# Autodesk Inventor assembly: vtx antanna pre assem 1
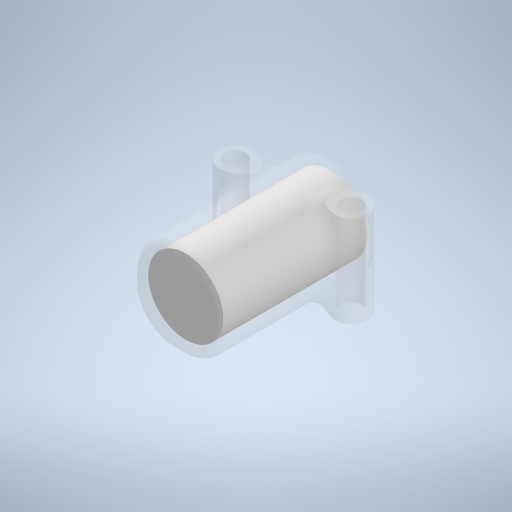
[picture p0: Inventor's stored thumbnail of the model, 512x512]
Saved by Autodesk Inventor 2023 (Build 270158000, 158)
## iProperties
Created: 2023-01-23
Part Number: vtx antanna pre assem 1
Document SubType Name: Assembly
Designer: Steven
Author: Steven
## Documents named in this file (4)
- Y:\FPV drone stuff\0 Street League\Frames\experimental-quad-frames\Nightstick MAX\3D prints\assems for derivs\vtx antanna pre assem 1.iam
- Y:\FPV drone stuff\0 Street League\Frames\experimental-quad-frames\Nightstick MAX\quad parts\SMA whip end.ipt
- Y:\FPV drone stuff\0 Street League\Frames\experimental-quad-frames\Nightstick MAX\3D prints\4700uF cap holder.ipt
- Y:\FPV drone stuff\0 Street League\Frames\experimental-quad-frames\Nightstick MAX\quad parts\4700uF cap.ipt
## Components (3 placed, 3 different names)
1. SMA whip end:1 — Mate:1, Flush:1, Flush:2, Flush:3, Angle:1
2. 4700uF cap holder:1 — Mate:1, Angle:1, Mate:2, Mate:3
3. 4700uF cap:1 — Mate:2, Mate:3
## Relationships (7: Mate 3, Flush 3, Angle 1)
- Mate:1: SMA whip end:1 ↔ 4700uF cap holder:1
- Flush:1: SMA whip end:1
- Flush:2: SMA whip end:1
- Flush:3: SMA whip end:1
- Angle:1 (0 deg): SMA whip end:1 ↔ 4700uF cap holder:1
- Mate:2: 4700uF cap holder:1 ↔ 4700uF cap:1
- Mate:3: 4700uF cap holder:1 ↔ 4700uF cap:1
